# Autodesk Inventor assembly: CameraUnit
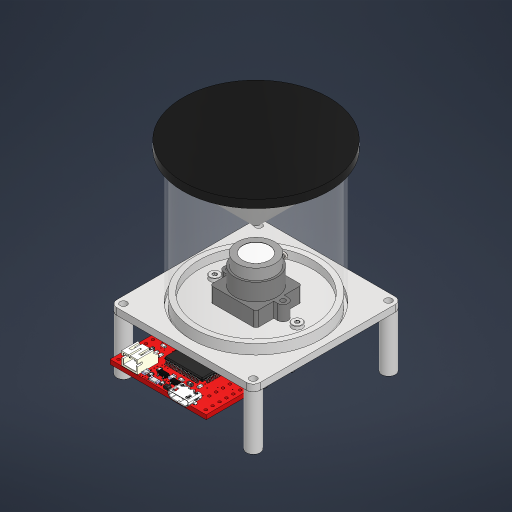
[picture p0: Inventor's stored thumbnail of the model, 512x512]
Saved by Autodesk Inventor 2024.2 (Build 282272000, 272)
## iProperties
Created: 2023-12-21
Part Number: CameraUnit
Document SubType Name: Assembly
Designer: Hanaoka
Author: Hanaoka
## Documents named in this file (7)
- G:\共有ドライブ\reRo\05_個人\hanaoka\inventor\CameraUnit\CameraUnit.iam
- G:\共有ドライブ\reRo\05_個人\hanaoka\inventor\CameraUnit\Camera_pipe.ipt
- G:\共有ドライブ\reRo\05_個人\hanaoka\inventor\CameraUnit\Camera_mirror.ipt
- G:\共有ドライブ\reRo\05_個人\hanaoka\inventor\CameraUnit\OpenMV_H7\OpenMV_H7.iam
- G:\共有ドライブ\reRo\05_個人\hanaoka\inventor\Screw\M2xL6\M2x6.ipt
- G:\共有ドライブ\reRo\05_個人\hanaoka\inventor\Spacer\Spacer_M2.6x20.ipt
- C:\Users\Hanaoka\Documents\Camera_Mount.ipt
## Components (10 placed, 6 different names)
1. Camera_pipe:1 — 挿入:2
2. Camera_mirror:1 — 挿入:2
3. OpenMV_H7:1 [sub-assembly] — フラッシュ:1
4. M2x6:1
5. M2x6:2
6. Spacer_M2.6x20:1
7. Spacer_M2.6x20:2
8. Spacer_M2.6x20:3
9. Spacer_M2.6x20:4
10. Camera_Mount:1 — フラッシュ:1
## Relationships (2: Insert 1, Flush 1)
- 挿入:2 [Insert]: Camera_pipe:1 ↔ Camera_mirror:1
- フラッシュ:1 [Flush]: OpenMV_H7:1 ↔ Camera_Mount:1
